# Autodesk Inventor assembly: Ankle_side_pitch
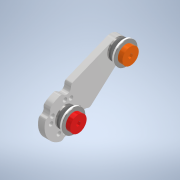
[picture p0: Inventor's stored thumbnail of the model, 180x180]
Saved by Autodesk Inventor 2020.4 (Build 244396000, 396)
## iProperties
Created: 2021-10-01
Part Number: Ankle_side_pitch
Document SubType Name: Assembly
Designer: Masato
Author: Masato
## Documents named in this file (10)
- C:\Users\Masato\Documents\Inventor\CIT Brains_Inventor\SUSTAINA-OP\LowerBody\Ankle\Ankle_side_pitch.iam
- C:\Users\Masato\Documents\Inventor\CIT Brains_Inventor\SUSTAINA-OP\LowerBody\Ankle\Ankle_side_pitch_frame.ipt
- C:\Users\Masato\Documents\Inventor\CIT Brains_Inventor\SUSTAINA-OP\ReadyMade\Bush\80F-0603.ipt
- C:\Users\Masato\Documents\Inventor\CIT Brains_Inventor\SUSTAINA-OP\ReadyMade\InsertNut\S4-05-3W.ipt
- C:\Users\Masato\Documents\Inventor\CIT Brains_Inventor\SUSTAINA-OP\ReadyMade\InsertNut\SF419.ipt
- C:\Users\Masato\Documents\Inventor\CIT Brains_Inventor\SUSTAINA-OP\ReadyMade\Washer\UUW-0412-10H.ipt
- C:\Users\Masato\Documents\Inventor\CIT Brains_Inventor\SUSTAINA-OP\ReadyMade\Washer\UUW-0614-05H.ipt
- C:\Users\Masato\Documents\Inventor\CIT Brains_Inventor\SUSTAINA-OP\ReadyMade\Screw\DBTS4-4.5-5-DHC-LTC_mod.ipt
- C:\Users\Masato\Documents\Inventor\CIT Brains_Inventor\SUSTAINA-OP\ReadyMade\Screw\DBTS4-4.5-5-DHC-LTC.ipt
- C:\Users\Masato\Documents\Inventor\CIT Brains_Inventor\SUSTAINA-OP\ReadyMade\Washer\TT-0814-10.ipt
## Components (13 placed, 9 different names)
1. Ankle_side_pitch_frame:1 — メイト:1, メイト:2, 角度:1, 挿入:1, 角度:2, 挿入:2, 挿入:3, 挿入:4
2. 80F-0603:1 — 挿入:5
3. 80F-0603:2 — 挿入:6
4. SF419:1 — 挿入:1
5. S4-05-3W:1 — 角度:2, 挿入:2
6. UUW-0412-10BH:1 — 挿入:3, 挿入:5, 挿入:7
7. UUW-0412-10BH:2 — 挿入:4, 挿入:6, 挿入:8
8. UUW-0614-05BH:1 — 挿入:9, 挿入:11
9. UUW-0614-05BH:2 — 挿入:10, 挿入:12
10. DBTS4-4.5-5-LTC_mod:1 — 挿入:7, 挿入:9
11. DBTS4-4.5-5-LTC:1 — 挿入:8, 挿入:10
12. TT-0814-10:1 — 挿入:11
13. TT-0814-10:2 — 挿入:12
## Relationships (16: Insert 12, Mate 2, Angle 2)
- メイト:1 [Mate]: Ankle_side_pitch_frame:1
- メイト:2 [Mate]: Ankle_side_pitch_frame:1
- 角度:1 [Angle] (147.9946 deg): Ankle_side_pitch_frame:1
- 挿入:1 [Insert]: Ankle_side_pitch_frame:1 ↔ SF419:1
- 角度:2 [Angle] (0 deg): Ankle_side_pitch_frame:1 ↔ S4-05-3W:1
- 挿入:2 [Insert]: Ankle_side_pitch_frame:1 ↔ S4-05-3W:1
- 挿入:3 [Insert]: Ankle_side_pitch_frame:1 ↔ UUW-0412-10BH:1
- 挿入:4 [Insert]: Ankle_side_pitch_frame:1 ↔ UUW-0412-10BH:2
- 挿入:5 [Insert]: 80F-0603:1 ↔ UUW-0412-10BH:1
- 挿入:6 [Insert]: 80F-0603:2 ↔ UUW-0412-10BH:2
- 挿入:7 [Insert]: UUW-0412-10BH:1 ↔ DBTS4-4.5-5-LTC_mod:1
- 挿入:8 [Insert]: UUW-0412-10BH:2 ↔ DBTS4-4.5-5-LTC:1
- 挿入:9 [Insert]: UUW-0614-05BH:1 ↔ DBTS4-4.5-5-LTC_mod:1
- 挿入:10 [Insert]: UUW-0614-05BH:2 ↔ DBTS4-4.5-5-LTC:1
- 挿入:11 [Insert]: UUW-0614-05BH:1 ↔ TT-0814-10:1
- 挿入:12 [Insert]: UUW-0614-05BH:2 ↔ TT-0814-10:2
